# Autodesk Inventor assembly: Final Assembly Jaden
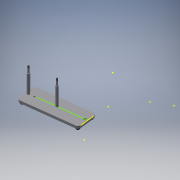
[picture p0: Inventor's stored thumbnail of the model, 180x180]
Saved by Autodesk Inventor 2017 (Build 210142000, 142)
## iProperties
Created: 2017-04-26
Part Number: Final Assembly Jaden
Document SubType Name: Assembly
Designer: 167898
Author: 167898
## Documents named in this file (5)
- C:\Users\167898.FCBOE\Documents\Final Assembly Jaden.iam
- C:\Users\167898.FCBOE\Downloads\Base Plate..ipt
- C:\Users\167898.FCBOE\Downloads\Rubber Foot..ipt
- C:\Users\167898.FCBOE\Downloads\screw.ipt
- C:\Users\167898.FCBOE\Downloads\Vertical Support..ipt
## Components (11 placed, 4 different names)
1. Base Plate.:1 — Rotational:1, Rotational:3, Rotational:4, Rotational:5, Rotational:6, Rigid:1
2. Rubber Foot.:1 — Rotational:4, Rotational:7
3. Rubber Foot.:2 — Rotational:5, Rotational:10
4. Rubber Foot.:3 — Rotational:3, Rotational:8
5. Rubber Foot.:4 — Rotational:6, Rotational:9
6. screw:1 — Rotational:8
7. screw:2 — Rotational:10
8. screw:3 — Rotational:7
9. screw:4 — Rotational:9
10. Vertical Support.:2 — Rotational:1
11. Vertical Support.:3 — Rigid:1
## Relationships (10: RevoluteJoint 9, WeldJoint 1)
- Rotational:1 [RevoluteJoint]: Base Plate.:1 ↔ Vertical Support.:2
- Rotational:3 [RevoluteJoint]: Base Plate.:1 ↔ Rubber Foot.:3
- Rotational:4 [RevoluteJoint]: Base Plate.:1 ↔ Rubber Foot.:1
- Rotational:5 [RevoluteJoint]: Base Plate.:1 ↔ Rubber Foot.:2
- Rotational:6 [RevoluteJoint]: Base Plate.:1 ↔ Rubber Foot.:4
- Rotational:7 [RevoluteJoint]: Rubber Foot.:1 ↔ screw:3
- Rotational:8 [RevoluteJoint]: Rubber Foot.:3 ↔ screw:1
- Rotational:9 [RevoluteJoint]: Rubber Foot.:4 ↔ screw:4
- Rotational:10 [RevoluteJoint]: Rubber Foot.:2 ↔ screw:2
- Rigid:1 [WeldJoint]: Base Plate.:1 ↔ Vertical Support.:3
